# Autodesk Inventor assembly: Assembly_All
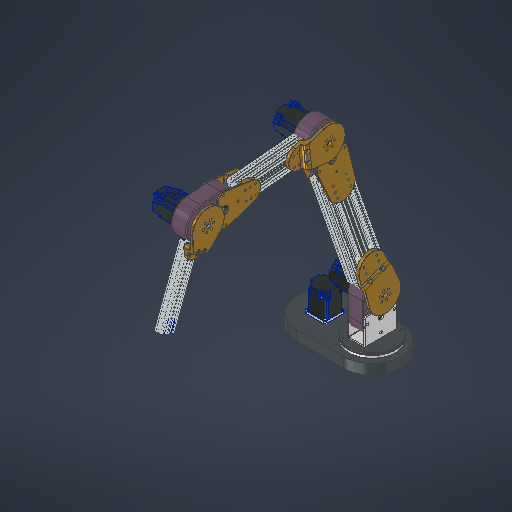
[picture p0: Inventor's stored thumbnail of the model, 512x512]
Saved by Autodesk Inventor 2026 (Build 300175000, 175)
## iProperties
RuleStatus: InUse
Created: 2025-11-30
Part Number: Assembly_All
Document SubType Name: Assembly
Designer: pochi
Author: pochi
## Documents named in this file (5)
- D:\POLIMI\3RD SEMESTER\Industrial Robotics\Project\Mine\Assembly_All.iam
- D:\POLIMI\3RD SEMESTER\Industrial Robotics\Project\Mine\Link_01_Assembly.iam
- D:\POLIMI\3RD SEMESTER\Industrial Robotics\Project\Mine\Link_02_Assembly.iam
- D:\POLIMI\3RD SEMESTER\Industrial Robotics\Project\Mine\Link_03_Assembly.iam
- D:\POLIMI\3RD SEMESTER\Industrial Robotics\Project\Mine\Base_Assembly.iam
## Components (4 placed, 4 different names)
1. Link_01_Assembly:1 [sub-assembly] — Mate:2, Cylindrical:1, Mate:4, Cylindrical:3
2. Link_02_Assembly:1 [sub-assembly] — Mate:2, Cylindrical:1, Mate:3, Cylindrical:2
3. Link_03_Assembly:1 [sub-assembly] — Mate:3, Cylindrical:2
4. Base_Assembly:1 [sub-assembly] — Mate:4, Cylindrical:3
## Relationships (6: Mate 3, CylindricalJoint 3)
- Mate:2: Link_01_Assembly:1 ↔ Link_02_Assembly:1
- Cylindrical:1: Link_01_Assembly:1 ↔ Link_02_Assembly:1
- Mate:3: Link_02_Assembly:1 ↔ Link_03_Assembly:1
- Cylindrical:2: Link_02_Assembly:1 ↔ Link_03_Assembly:1
- Mate:4: Link_01_Assembly:1 ↔ Base_Assembly:1
- Cylindrical:3: Link_01_Assembly:1 ↔ Base_Assembly:1
